# Autodesk Inventor assembly: tower
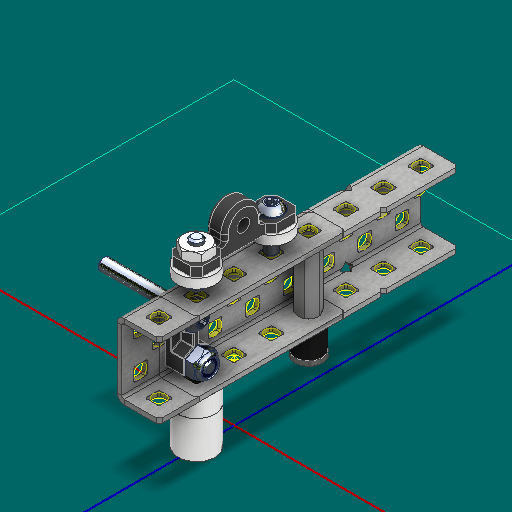
[picture p0: Inventor's stored thumbnail of the model, 512x512]
Saved by Autodesk Inventor 2025 (Build 290162000, 162)
## iProperties
Created: 2024-08-17
Part Number: tower
Document SubType Name: Assembly
Designer: averey
Author: averey
## Documents named in this file (20)
- C:\Users\avere\vex_robotics_high_stakes\hardware\cad\ATLAS\intake\first_stage\tower.iam
- C:\Users\avere\vex_robotics_high_stakes\hardware\cad\VEX-CAD-Inventor\Structure\C Channel\Aluminum 1x2x1\Alu C 1x2x1x5.ipt
- C:\Users\avere\vex_robotics_high_stakes\hardware\cad\VEX-CAD-Inventor\Motion\Spacers\Spacer Nylon .375 OD.ipt
- C:\Users\avere\vex_robotics_high_stakes\hardware\cad\VEX-CAD-Inventor\Motion\Spacers\Washer Steel\SWasher .375 OD x .062500.ipt
- C:\Users\avere\vex_robotics_high_stakes\hardware\cad\VEX-CAD-Inventor\Motion\Spacers\Washer Steel.ipt
- C:\Users\avere\vex_robotics_high_stakes\hardware\cad\VEX-CAD-Inventor\Motion\Spacers\Spacer Nylon .500 OD\NSpacer White .500 OD x .250.ipt
- C:\Users\avere\vex_robotics_high_stakes\hardware\cad\VEX-CAD-Inventor\Motion\Spacers\Spacer Nylon .500 OD.ipt
- C:\Users\avere\vex_robotics_high_stakes\hardware\cad\VEX-CAD-Inventor\Motion\Spacers\Spacer Nylon .500 OD\NSpacer White .500 OD x .500.ipt
- C:\Users\avere\vex_robotics_high_stakes\hardware\cad\VEX-CAD-Inventor\Structure\Standoff\Standoff .875.ipt
- C:\Users\avere\vex_robotics_high_stakes\hardware\cad\VEX-CAD-Inventor\Structure\Standoff.ipt
- C:\Users\avere\vex_robotics_high_stakes\hardware\cad\VEX-CAD-Inventor\Structure\C Channel\Aluminum 1x2x1\Alu C 1x2x1x4.ipt
- C:\Users\avere\vex_robotics_high_stakes\hardware\cad\ATLAS\intake\first_stage\top_roller_bearing.iam
- C:\Users\avere\vex_robotics_high_stakes\hardware\cad\custom_parts\modified_parts\Bearing Flat Low Profile 2-Hole.ipt
- C:\Users\avere\vex_robotics_high_stakes\hardware\cad\VEX-CAD-Inventor\Structure\Hardware\Screw Steel - Star\SScrew Star Smooth 1.250.ipt
- C:\Users\avere\vex_robotics_high_stakes\hardware\cad\VEX-CAD-Inventor\Structure\Hardware\Screw Steel - Star.ipt
- C:\Users\avere\vex_robotics_high_stakes\hardware\cad\VEX-CAD-Inventor\Structure\Hardware\Screw Shoulder Robosource\SScrew Shoulder Smooth .500 x .04.ipt
- C:\Users\avere\vex_robotics_high_stakes\hardware\cad\VEX-CAD-Inventor\Structure\Hardware\Screw Shoulder Robosource.ipt
- C:\Users\avere\vex_robotics_high_stakes\hardware\cad\VEX-CAD-Inventor\Structure\Hardware\Nut Thin Nylock.ipt
- C:\Users\avere\vex_robotics_high_stakes\hardware\cad\VEX-CAD-Inventor\Motion\Spacers\Spacer Nylon .375 OD\NSpacer .375 OD x .375.ipt
- C:\Users\avere\vex_robotics_high_stakes\hardware\cad\VEX-CAD-Inventor\Structure\C Channel\Aluminum 1x2x1\Alu C 1x2x1x7.ipt
## Components (13 placed, 13 different names)
1. Alu C 1x2x1x5:1 — Mate:1, Insert:6, Insert:7, Mate:2
2. SWasher .375 OD x .062500:1 — Insert:15
3. NSpacer White .500 OD x .250:1 — Insert:8
4. NSpacer White .500 OD x .500:2
5. Standoff .875:1 — Insert:6
6. Alu C 1x2x1x4:1 — Insert:7, Mate:2, Insert:8, Insert:13, Mate:4, Insert:14, Insert:17, Mate:6, Insert:18, Mate:7
7. top_roller_bearing:1 [sub-assembly] — Insert:18, Mate:7
8. Bearing Flat Low Profile 2-Hole:1 — Insert:10, Insert:11, Insert:12
9. SScrew Star Smooth 1.250:1 — Insert:10, Mate:4
10. SScrew Shoulder Smooth .500 x .04:1 — Insert:11, Insert:13
11. Nut Thin Nylock:1 — Insert:12
12. NSpacer .375 OD x .375:1 — Insert:14, Insert:15
13. Alu C 1x2x1x7:1 — Insert:17, Mate:6
## Relationships (17: Insert 12, Mate 5)
- [Insert]: NSpacer White .500 OD x .250:1 ↔ NSpacer White .500 OD x .500:2
- Mate:1: Alu C 1x2x1x5:1
- Insert:6: Alu C 1x2x1x5:1 ↔ Standoff .875:1
- Insert:7: Alu C 1x2x1x5:1 ↔ Alu C 1x2x1x4:1
- Mate:2: Alu C 1x2x1x5:1 ↔ Alu C 1x2x1x4:1
- Insert:8: NSpacer White .500 OD x .250:1 ↔ Alu C 1x2x1x4:1
- Insert:10 (1.27 mm): Bearing Flat Low Profile 2-Hole:1 ↔ SScrew Star Smooth 1.250:1
- Insert:11 (1.5875 mm): Bearing Flat Low Profile 2-Hole:1 ↔ SScrew Shoulder Smooth .500 x .04:1
- Insert:12 (1.27 mm): Bearing Flat Low Profile 2-Hole:1 ↔ Nut Thin Nylock:1
- Insert:13: Alu C 1x2x1x4:1 ↔ SScrew Shoulder Smooth .500 x .04:1
- Mate:4: Alu C 1x2x1x4:1 ↔ SScrew Star Smooth 1.250:1
- Insert:14: Alu C 1x2x1x4:1 ↔ NSpacer .375 OD x .375:1
- Insert:15: SWasher .375 OD x .062500:1 ↔ NSpacer .375 OD x .375:1
- Insert:17: Alu C 1x2x1x4:1 ↔ Alu C 1x2x1x7:1
- Mate:6: Alu C 1x2x1x4:1 ↔ Alu C 1x2x1x7:1
- Insert:18 (6.35 mm): Alu C 1x2x1x4:1 ↔ top_roller_bearing:1
- Mate:7: Alu C 1x2x1x4:1 ↔ top_roller_bearing:1
